# Autodesk Inventor assembly: marker release
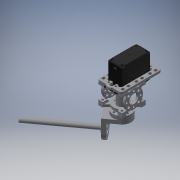
[picture p0: Inventor's stored thumbnail of the model, 180x180]
Saved by Autodesk Inventor 2019 (Build 230136000, 136)
## iProperties
Created: 2018-11-20
Part Number: marker release
Document SubType Name: Assembly
Designer: User
Author: User
## Documents named in this file (5)
- C:\Robotics\CAD\2018-19_CAD\marker release.iam
- C:\Robotics\CAD\2018-19_CAD\smart servo with servo block.iam
- C:\Robotics\CAD\COTSParts\Actobotics\545 parts\545400PatternMount90degrees.ipt
- C:\Robotics\CAD\COTSParts\Actobotics\535 parts\535198Bearing.25ID.5OD.ipt
- C:\Robotics\CAD\COTSParts\Actobotics\634 parts\634078.25inDShaft3.5inLong.ipt
## Components (4 placed, 4 different names)
1. smart servo with servo block:1 [sub-assembly] — Mate:1, Mate:2, Mate:3
2. 545400PatternMount90degrees:1 — Mate:1, Mate:2, Mate:3, Mate:4, Mate:5, Flush:1
3. 535198Bearing.25ID.5OD:1 — Mate:4, Mate:5, Mate:6
4. 634078.25inDShaft3.5inLong:1 — Mate:6, Flush:1
## Relationships (7: Mate 6, Flush 1)
- Mate:1: smart servo with servo block:1 ↔ 545400PatternMount90degrees:1
- Mate:2: smart servo with servo block:1 ↔ 545400PatternMount90degrees:1
- Mate:3: smart servo with servo block:1 ↔ 545400PatternMount90degrees:1
- Mate:4: 545400PatternMount90degrees:1 ↔ 535198Bearing.25ID.5OD:1
- Mate:5: 545400PatternMount90degrees:1 ↔ 535198Bearing.25ID.5OD:1
- Mate:6: 535198Bearing.25ID.5OD:1 ↔ 634078.25inDShaft3.5inLong:1
- Flush:1: 545400PatternMount90degrees:1 ↔ 634078.25inDShaft3.5inLong:1
